# Autodesk Inventor assembly: 付け根_1
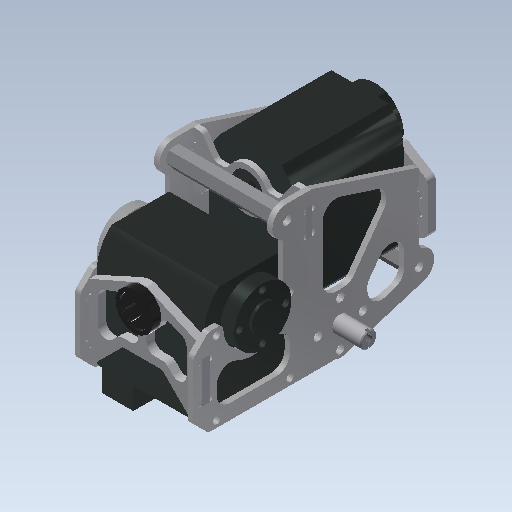
[picture p0: Inventor's stored thumbnail of the model, 512x512]
Saved by Autodesk Inventor 2020 (Build 240168000, 168)
## iProperties
Created: 2016-04-27
Part Number: 付け根_1
Document SubType Name: Assembly
Designer: hiroaki
Mass: 257.123 g
Surface Area: 430.699 cm^2
Volume: 127.027 cm^3
Density: 2.02416 g/cm^3
Author: hiroaki
## Documents named in this file (13)
- C:\Users\Masato\Documents\Inventor\CIT Brains_Inventor\OpenPlatform_ver3_0\下半身_160823\付け根\付け根_1.iam
- C:\Users\Masato\Documents\Inventor\CIT Brains_Inventor\OpenPlatform_ver3_0\既製品\B3M11xx.ipt
- C:\Users\Masato\Documents\Inventor\CIT Brains_Inventor\OpenPlatform_ver3_0\既製品\free_horn.ipt
- C:\Users\Masato\Documents\Inventor\CIT Brains_Inventor\OpenPlatform_ver3_0\下半身_160823\付け根\付け根_サブフレーム_1_2.ipt
- C:\Users\Masato\Documents\Inventor\CIT Brains_Inventor\OpenPlatform_ver3_0\既製品\BRU-305_5.ipt
- C:\Users\Masato\Documents\Inventor\CIT Brains_Inventor\OpenPlatform_ver3_0\下半身_160823\付け根\付け根_サブフレーム_6_2.ipt
- C:\Users\Masato\Documents\Inventor\CIT Brains_Inventor\OpenPlatform_ver3_0\下半身_160823\付け根\付け根_サブフレーム_1_4.ipt
- C:\Users\Masato\Documents\Inventor\CIT Brains_Inventor\OpenPlatform_ver3_0\下半身_160823\付け根\付け根_メインフレーム_2_1.ipt
- C:\Users\Masato\Documents\Inventor\CIT Brains_Inventor\OpenPlatform_ver3_0\下半身_160823\付け根\付け根_サブフレーム_1_3.ipt
- C:\Users\Masato\Documents\Inventor\CIT Brains_Inventor\OpenPlatform_ver3_0\下半身_160823\付け根\付け根_メインフレーム_6_1.ipt
- C:\Users\Masato\Documents\Inventor\CIT Brains_Inventor\OpenPlatform_ver3_0\既製品\SLSBF6-39_5-M3-N3.ipt
- C:\Users\Masato\Documents\Inventor\CIT Brains_Inventor\OpenPlatform_ver3_0\既製品\新規購入\BRU-312.5S.ipt
- C:\Users\Masato\Documents\Inventor\CIT Brains_Inventor\OpenPlatform_ver3_0\既製品\新規購入\FFW-0312-20B.ipt
## Components (17 placed, 12 different names)
1. free_horn:1 — 挿入:1
2. B3M11xx:3 — 挿入:1, 挿入:63, 挿入:64, メイト:18, 挿入:77, 挿入:78
3. B3M11xx:4 — 挿入:7, 挿入:8, 挿入:74, 挿入:75
4. 付け根_サブフレーム_1_2:1 — 挿入:7, 挿入:8, メイト:16, フラッシュ:1, メイト:22
5. BRU-305_5:1 — 挿入:52, 挿入:76
6. 付け根_サブフレーム_1_4:1 — 挿入:82
7. 付け根_サブフレーム_6_2:1 — 挿入:52
8. 付け根_メインフレーム_2_1:1 — 挿入:63, 挿入:64, メイト:16, メイト:20, フラッシュ:1, メイト:21, メイト:22, 挿入:83, 挿入:84, 挿入:85, 挿入:88
9. 付け根_サブフレーム_1_3:1 — メイト:18, メイト:20, メイト:21, 挿入:82
10. 付け根_メインフレーム_6_1:1 — 挿入:74, 挿入:75, 挿入:76
11. 付け根_メインフレーム_2_1:2 — 挿入:77, 挿入:78, 挿入:86, 挿入:87
12. SLSBF6-39_5-M3-N3:1 — 挿入:83
13. SLSBF6-39_5-M3-N3:2 — 挿入:84
14. BRU-312.5S:1 — 挿入:85
15. BRU-312.5S:2 — 挿入:86
16. FFW-0312-20B:1 — 挿入:88
17. FFW-0312-20B:2 — 挿入:87
## Relationships (24: Insert 18, Mate 5, Flush 1)
- 挿入:1 [Insert]: free_horn:1 ↔ B3M11xx:3
- 挿入:7 [Insert]: B3M11xx:4 ↔ 付け根_サブフレーム_1_2:1
- 挿入:8 [Insert]: B3M11xx:4 ↔ 付け根_サブフレーム_1_2:1
- 挿入:52 [Insert]: BRU-305_5:1 ↔ 付け根_サブフレーム_6_2:1
- 挿入:63 [Insert]: B3M11xx:3 ↔ 付け根_メインフレーム_2_1:1
- 挿入:64 [Insert]: B3M11xx:3 ↔ 付け根_メインフレーム_2_1:1
- メイト:16 [Mate]: 付け根_サブフレーム_1_2:1 ↔ 付け根_メインフレーム_2_1:1
- フラッシュ:1 [Flush]: 付け根_サブフレーム_1_2:1 ↔ 付け根_メインフレーム_2_1:1
- メイト:18 [Mate]: B3M11xx:3 ↔ 付け根_サブフレーム_1_3:1
- メイト:20 [Mate] (0.01 mm): 付け根_メインフレーム_2_1:1 ↔ 付け根_サブフレーム_1_3:1
- 挿入:74 [Insert]: B3M11xx:4 ↔ 付け根_メインフレーム_6_1:1
- 挿入:75 [Insert]: B3M11xx:4 ↔ 付け根_メインフレーム_6_1:1
- 挿入:76 [Insert]: BRU-305_5:1 ↔ 付け根_メインフレーム_6_1:1
- メイト:21 [Mate]: 付け根_メインフレーム_2_1:1 ↔ 付け根_サブフレーム_1_3:1
- メイト:22 [Mate] (0.01 mm): 付け根_サブフレーム_1_2:1 ↔ 付け根_メインフレーム_2_1:1
- 挿入:77 [Insert]: B3M11xx:3 ↔ 付け根_メインフレーム_2_1:2
- 挿入:78 [Insert]: B3M11xx:3 ↔ 付け根_メインフレーム_2_1:2
- 挿入:82 [Insert]: 付け根_サブフレーム_1_4:1 ↔ 付け根_サブフレーム_1_3:1
- 挿入:83 [Insert]: 付け根_メインフレーム_2_1:1 ↔ SLSBF6-39_5-M3-N3:1
- 挿入:84 [Insert]: 付け根_メインフレーム_2_1:1 ↔ SLSBF6-39_5-M3-N3:2
- 挿入:85 [Insert]: 付け根_メインフレーム_2_1:1 ↔ BRU-312.5S:1
- 挿入:86 [Insert]: 付け根_メインフレーム_2_1:2 ↔ BRU-312.5S:2
- 挿入:87 [Insert]: 付け根_メインフレーム_2_1:2 ↔ FFW-0312-20B:2
- 挿入:88 [Insert]: 付け根_メインフレーム_2_1:1 ↔ FFW-0312-20B:1
